# Autodesk Inventor assembly: Coupler bottom fixed + pulleys
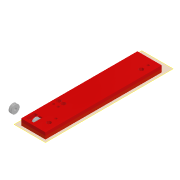
[picture p0: Inventor's stored thumbnail of the model, 180x180]
Saved by Autodesk Inventor 2020 (Build 240168000, 168)
## iProperties
Created: 2019-11-17
Part Number: Coupler bottom fixed + pulleys
Document SubType Name: Assembly
Designer: ball
Author: ball
## Documents named in this file (3)
- C:\FTC\FTC8863CAD\2019 Robot\Delivery\Coupler bottom fixed + pulleys.iam
- C:\FTC\FTC8863CAD\2019 Robot\Delivery\Coupler bottom fixed.ipt
- C:\FTC\FTC8863CAD\RevRobotics\REV-41-1368 pulley.ipt
## Components (3 placed, 2 different names)
1. Coupler bottom fixed:1 — Mate:3, Mate:4
2. REV-41-1368 pulley:1 — Mate:3, Mate:4
3. REV-41-1368 pulley:2
## Relationships (2: Mate 2)
- Mate:3: Coupler bottom fixed:1 ↔ REV-41-1368 pulley:1
- Mate:4: Coupler bottom fixed:1 ↔ REV-41-1368 pulley:1
